# Autodesk Inventor assembly: Claw_1
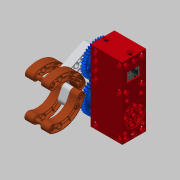
[picture p0: Inventor's stored thumbnail of the model, 180x180]
Saved by Autodesk Inventor 2019.3 (Build 233278000, 278)
## iProperties
Created: 2019-03-18
Part Number: Claw_1
Document SubType Name: Assembly
Designer: Varga Daniel
Author: Varga Daniel
## Documents named in this file (8)
- C:\!_Dani\!_cloud\OneDrive\!_munka\Revolution\RevvyDemoKit\Structural parts\Test assemblies\Claw_small_3_double.iam
- C:\!_Dani\!_cloud\OneDrive\!_munka\Revolution\RevvyDemoKit\Structural parts\Connetor Pins\CP1+x1+\CP1x1.ipt
- C:\!_Dani\!_cloud\OneDrive\!_munka\Revolution\RevvyDemoKit\Structural parts\Gears\G40.ipt
- C:\!_Dani\!_cloud\OneDrive\!_munka\Revolution\RevvyDemoKit\Structural parts\Demo parts\Motor\Inventor imported\motor.iam
- C:\!_Dani\!_cloud\OneDrive\!_munka\Revolution\RevvyDemoKit\Structural parts\Axles\AXp2p.ipt
- C:\!_Dani\!_cloud\OneDrive\!_munka\Revolution\RevvyDemoKit\Structural parts\Beams\Straight Beams\S2+x2\S4x2.ipt
- C:\!_Dani\!_cloud\OneDrive\!_munka\Revolution\RevvyDemoKit\Structural parts\Beams\Curved beams\CB4H.ipt
- C:\!_Dani\!_cloud\OneDrive\!_munka\Revolution\RevvyDemoKit\Structural parts\Connetor Pins\CP1+x1+\CP2x1.ipt
## Components (21 placed, 7 different names)
1. CB4H:1 — Insert:29, Mate:10
2. G40:1 — Mate:6, Angle:1, Rotation:1, Insert:34, Insert:35, Insert:42
3. motor:1 [sub-assembly] — Mate:1, Flush:1, Mate:2, Insert:5, Mate:6, Angle:2
4. AXp2p:1 — Mate:3, Mate:4, Mate:5, Insert:5
5. G40:2 — Mate:3, Mate:4, Mate:5, Angle:1, Angle:2, Rotation:1, Insert:38, Insert:39
6. CB4H:2 — Mate:9, Insert:30
7. S4x2:1 — Insert:36, Insert:37
8. S4x2:2 — Insert:40, Insert:41
9. CP2x1:3 — Insert:31
10. CP2x1:2
11. CP2x1:4
12. CP2x1:5
13. CB4H:3 — Mate:10, Insert:32
14. CB4H:4 — Mate:9, Insert:31
15. CP2x1:6 — Insert:30
16. CP2x1:7 — Insert:29, Insert:32
17. CP1x1:9 — Insert:34, Insert:37
18. CP1x1:10 — Insert:39, Insert:40
19. CP1x1:11 — Insert:38, Insert:41
20. CP2x1:8 — Insert:35, Insert:36
21. CP1x1:12 — Insert:42
## Relationships (34: Insert 22, Mate 8, Angle 2, Flush 1, RelateRotation 1)
- Mate:1: motor:1
- Flush:1: motor:1
- Mate:2: motor:1
- Mate:3: AXp2p:1 ↔ G40:2
- Mate:4: AXp2p:1 ↔ G40:2
- Mate:5: AXp2p:1 ↔ G40:2
- Insert:5: motor:1 ↔ AXp2p:1
- Mate:6: G40:1 ↔ motor:1
- Angle:1 (0 deg): G40:1 ↔ G40:2
- Angle:2 (0 deg): motor:1 ↔ G40:2
- [Insert]: S4x2:1 ↔ CP2x1:3
- [Insert]: S4x2:1 ↔ CP2x1:2
- [Insert]: CB4H:2 ↔ CP2x1:3
- [Insert]: CB4H:2 ↔ CP2x1:2
- [Insert]: S4x2:2 ↔ CP2x1:4
- [Insert]: S4x2:2 ↔ CP2x1:5
- [Insert]: CB4H:1 ↔ CP2x1:4
- [Insert]: CB4H:1 ↔ CP2x1:5
- Rotation:1 [RelateRotation] (1 ul): G40:1 ↔ G40:2
- Insert:29: CB4H:1 ↔ CP2x1:7
- Mate:9: CB4H:2 ↔ CB4H:4
- Insert:30: CB4H:2 ↔ CP2x1:6
- Insert:31: CP2x1:3 ↔ CB4H:4
- Mate:10: CB4H:1 ↔ CB4H:3
- Insert:32: CB4H:3 ↔ CP2x1:7
- Insert:34: G40:1 ↔ CP1x1:9
- Insert:35: G40:1 ↔ CP2x1:8
- Insert:36: S4x2:1 ↔ CP2x1:8
- Insert:37: S4x2:1 ↔ CP1x1:9
- Insert:38: G40:2 ↔ CP1x1:11
- Insert:39: G40:2 ↔ CP1x1:10
- Insert:40: S4x2:2 ↔ CP1x1:10
- Insert:41: S4x2:2 ↔ CP1x1:11
- Insert:42: G40:1 ↔ CP1x1:12
